# Autodesk Inventor assembly: Zespół2
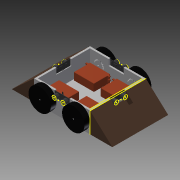
[picture p0: Inventor's stored thumbnail of the model, 180x180]
Saved by Autodesk Inventor 2014 (Build 180170000, 170)
## iProperties
Created: 2013-10-14
Part Number: Zespół2
Document SubType Name: Assembly
Designer: Wojciech
Author: Wojciech
## Documents named in this file (14)
- C:\Users\Wojciech\Desktop\sumo\Zespół2.iam
- C:\Users\Wojciech\Desktop\sumo\korpus.ipt
- C:\Users\Wojciech\Desktop\sumo\koło.ipt
- C:\Users\Wojciech\Desktop\sumo\Serwo.ipt
- C:\Users\Wojciech\Desktop\sumo\zebatka.ipt
- C:\Users\Wojciech\Desktop\sumo\os.ipt
- C:\Users\Wojciech\Desktop\sumo\czujnik_ultra_dzwiek.ipt
- C:\Users\Wojciech\Desktop\sumo\klin.ipt
- C:\Users\Wojciech\Desktop\sumo\Zespół2\AIP\FEA\aub14bmyo.fins
- C:\Users\Wojciech\Desktop\sumo\Zespół2\AIP\FEA\aub14bmyo.fsat
- C:\Users\Wojciech\Desktop\sumo\Zespół2\AIP\FEA\aub14bmyo.ftes
- C:\Users\Wojciech\Desktop\sumo\Zespół2\AIP\FEA\aub14bmyo.fwiz
- C:\Users\Wojciech\Desktop\sumo\Zespół2\AIP\FEA\aub14bmyp.fmsh
- C:\Users\Wojciech\Desktop\sumo\Zespół2\AIP\FEA\aub14bmyq.fres
## Components (23 placed, 7 different names)
1. korpus:1 — Obrotowe:9, Obrotowe:10, Obrotowe:11, Obrotowe:12, Zestawiający:1, Zestawiający:2, Zestawiający:3, Zestawiający:4, Sztywne:1, Sztywne:2
2. koło:1 — Obrotowe:9, Obrotowe:13
3. koło:2 — Obrotowe:7, Obrotowe:10, Obrotowe:14
4. koło:3 — Obrotowe:11, Obrotowe:15
5. koło:4 — Obrotowe:12, Obrotowe:16
6. Serwo:1
7. Serwo:2
8. Serwo:3
9. Serwo:4
10. zebatka:1 — Obrotowe:19
11. zebatka:2 — Obrotowe:18
12. zebatka:3 — Obrotowe:7
13. zebatka:4 — Obrotowe:17
14. os:1 — Obrotowe:15, Obrotowe:18
15. os:2 — Obrotowe:14
16. os:3 — Obrotowe:13, Obrotowe:17
17. os:4 — Obrotowe:16, Obrotowe:19
18. czujnik_ultra_dzwiek:1 — Zestawiający:3
19. czujnik_ultra_dzwiek:2 — Zestawiający:2
20. czujnik_ultra_dzwiek:3 — Zestawiający:4
21. czujnik_ultra_dzwiek:4 — Zestawiający:1
22. klin:1 — Sztywne:2
23. klin:2 — Sztywne:1
## Relationships (18: RevoluteJoint 12, Mate 4, WeldJoint 2)
- Obrotowe:7 [RevoluteJoint] (5 mm): koło:2 ↔ zebatka:3
- Obrotowe:9 [RevoluteJoint] (15 mm): korpus:1 ↔ koło:1
- Obrotowe:10 [RevoluteJoint]: korpus:1 ↔ koło:2
- Obrotowe:11 [RevoluteJoint]: korpus:1 ↔ koło:3
- Obrotowe:12 [RevoluteJoint]: korpus:1 ↔ koło:4
- Obrotowe:13 [RevoluteJoint] (5 mm): koło:1 ↔ os:3
- Obrotowe:14 [RevoluteJoint] (-5 mm): koło:2 ↔ os:2
- Obrotowe:15 [RevoluteJoint] (5 mm): koło:3 ↔ os:1
- Obrotowe:16 [RevoluteJoint] (-5 mm): koło:4 ↔ os:4
- Obrotowe:17 [RevoluteJoint] (-3 mm): zebatka:4 ↔ os:3
- Obrotowe:18 [RevoluteJoint] (-3 mm): zebatka:2 ↔ os:1
- Obrotowe:19 [RevoluteJoint] (-3 mm): zebatka:1 ↔ os:4
- Zestawiający:1 [Mate] (-2 mm): korpus:1 ↔ czujnik_ultra_dzwiek:4
- Zestawiający:2 [Mate]: korpus:1 ↔ czujnik_ultra_dzwiek:2
- Zestawiający:3 [Mate]: korpus:1 ↔ czujnik_ultra_dzwiek:1
- Zestawiający:4 [Mate] (2 mm): korpus:1 ↔ czujnik_ultra_dzwiek:3
- Sztywne:1 [WeldJoint]: korpus:1 ↔ klin:2
- Sztywne:2 [WeldJoint]: korpus:1 ↔ klin:1
## Named parameters: sa_0 = -2000, sa_1 = 0, sa_2 = 0, sa_3 = 2000, sa_4 = 0, sa_5 = 0
note: some values were not read from the file. Shown as the stored number, unit unknown: "sa_0", "sa_1", "sa_2", "sa_3", "sa_4", "sa_5".
